# Autodesk Inventor assembly: main climber
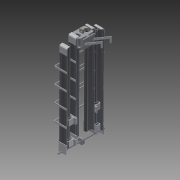
[picture p0: Inventor's stored thumbnail of the model, 180x180]
Saved by Autodesk Inventor 2013 (Build 170138000, 138)
## iProperties
Created: 2013-01-25
Part Number: main climber
Document SubType Name: Assembly
Designer: Arpan
Mass: 3339.77 g
Surface Area: 12818.3 cm^2
Volume: 2944.87 cm^3
Density: 1.1341 g/cm^3
Author: Arpan
## Documents named in this file (16)
- C:\Users\Moses\Documents\GitHub\frc2013CAD\Cimber actual\main climber.iam
- C:\Users\Moses\Documents\GitHub\frc2013CAD\Cimber actual\Shaft 26 inch.ipt
- C:\Users\Moses\Documents\GitHub\frc2013CAD\Cimber actual\Bearing Block long style.iam
- C:\Users\Moses\Documents\GitHub\frc2013CAD\Cimber actual\hook mount plate.ipt
- C:\Users\Moses\Documents\GitHub\frc2013CAD\Cimber actual\tie-together tier 1.ipt
- C:\Users\Moses\Documents\GitHub\frc2013CAD\Cimber actual\endstop.ipt
- C:\Users\Moses\Documents\GitHub\frc2013CAD\Cimber actual\hook faceplate.ipt
- C:\Users\Moses\Documents\GitHub\frc2013CAD\Cimber actual\hook.ipt
- C:\Users\Moses\Documents\GitHub\frc2013CAD\Cimber actual\face mount.ipt
- C:\Users\Moses\Documents\GitHub\frc2013CAD\Cimber actual\bearing block short style.iam
- C:\Users\Moses\Documents\GitHub\frc2013CAD\Cimber actual\upper face mount.ipt
- C:\Users\Moses\Documents\GitHub\frc2013CAD\Cimber actual\tie-together tier 2.ipt
- C:\Users\Moses\Documents\GitHub\frc2013CAD\Cimber actual\arm mout.ipt
- C:\Users\Moses\Documents\GitHub\frc2013CAD\Cimber actual\14 inch shaft.ipt
- C:\Users\Moses\Documents\GitHub\frc2013CAD\Cimber actual\rough pulley.ipt
- C:\Users\Moses\Documents\GitHub\frc2013CAD\Cimber actual\hook mount plate 2.ipt
## Components (34 placed, 15 different names)
1. Shaft 26 inch:1 — Flush:1, Angle:1, Mate:2, Flush:2, Angle:2, Mate:12, Mate:13, Mate:25, Mate:26, Mate:27, Mate:28, Mate:29, Mate:30, Mate:31, Mate:32, Mate:33, Mate:38, Mate:39, Mate:40, Mate:46, Mate:53, Mate:54, Mate:55
2. Shaft 26 inch:2 — Flush:1, Angle:1, Mate:1, Flush:2, Flush:7, Mate:10, Mate:11, Mate:37, Flush:15, Flush:16, Mate:48, Mate:50, Mate:51, Mate:52
3. Bearing Block long style:1 [sub-assembly] — Mate:1, Mate:3, Flush:3
4. Bearing Block long style:2 [sub-assembly] — Mate:2, Mate:3, Angle:2, Flush:3, Mate:98, Flush:25, Flush:26
5. hook mount plate:1 — Mate:98, Mate:99, Flush:25, Flush:26, Flush:27, Mate:100, Flush:28, Mate:101, Flush:29
6. endstop:1 — Mate:12, Mate:13, Mate:46
7. endstop:2 — Flush:7, Mate:10, Mate:11
8. hook faceplate:1 — Mate:20, Mate:21, Mate:22, Flush:13, Flush:14, Mate:23, Mate:99, Mate:101, Flush:29, Mate:102, Flush:30
9. hook:1 — Mate:22, Flush:14, Mate:102
10. hook:2 — Mate:20, Mate:21, Flush:13, Mate:23
11. tie-together tier 1:1 — Mate:25, Mate:26, Mate:27
12. tie-together tier 1:2 — Mate:28, Mate:29, Mate:30
13. tie-together tier 1:3 — Mate:31, Mate:32, Mate:33
14. face mount:1 — Mate:37, Flush:15, Flush:16, Mate:43, Mate:84, Mate:85
15. face mount:2 — Mate:38, Mate:39, Mate:40, Flush:17, Mate:41, Flush:18
16. bearing block short style:1 [sub-assembly] — Flush:17, Mate:41, Flush:18
17. bearing block short style:2 [sub-assembly] — Mate:43, Flush:19, Mate:49, Mate:84, Mate:85, Flush:23
18. bearing block short style:3 [sub-assembly] — Mate:57, Mate:58, Mate:59, Mate:60, Mate:64, Angle:3
19. bearing block short style:4 [sub-assembly] — Mate:48, Flush:19, Mate:49, Mate:65
20. upper face mount:1 — Mate:50, Mate:51, Mate:52
21. upper face mount:2 — Mate:53, Mate:54, Mate:55, Mate:57, Mate:58, Mate:59, Mate:60
22. Shaft 26 inch:3 — Mate:65, Angle:4, Flush:20, Mate:67, Mate:68, Flush:22, Mate:78, Mate:79, Mate:80, Mate:82, Mate:83, Flush:23, Mate:88, Mate:89
23. Shaft 26 inch:4 — Mate:64, Angle:3, Angle:4, Flush:20, Mate:69, Mate:70, Mate:71, Mate:76, Mate:77, Mate:86, Mate:87, Mate:90, Mate:91, Mate:97
24. endstop:3 — Mate:67, Mate:68, Flush:22
25. endstop:4 — Mate:69, Mate:70, Mate:71
26. tie-together tier 2:2 — Mate:76, Mate:77, Mate:78
27. tie-together tier 2:3 — Mate:79, Mate:80
28. tie-together tier 2:4 — Mate:82, Mate:83
29. tie-together tier 2:5 — Mate:86, Mate:87
30. arm mout:1 — Mate:90, Mate:91, Mate:92, Mate:97
31. arm mout:2 — Mate:88, Mate:89, Flush:24, Mate:96
32. 14 inch shaft:1 — Mate:92, Flush:24, Mate:93
33. rough pulley:1 — Mate:93, Mate:96
34. hook mount plate 2:1 — Flush:27, Mate:100, Flush:28, Flush:30
## Relationships (95: Mate 70, Flush 21, Angle 4)
- Flush:1: Shaft 26 inch:1 ↔ Shaft 26 inch:2
- Angle:1 (180 deg): Shaft 26 inch:1 ↔ Shaft 26 inch:2
- Mate:1: Shaft 26 inch:2 ↔ Bearing Block long style:1
- Mate:2: Shaft 26 inch:1 ↔ Bearing Block long style:2
- Mate:3 (12.7 mm): Bearing Block long style:1 ↔ Bearing Block long style:2
- Flush:2: Shaft 26 inch:1 ↔ Shaft 26 inch:2
- Angle:2 (0 deg): Shaft 26 inch:1 ↔ Bearing Block long style:2
- Flush:3: Bearing Block long style:1 ↔ Bearing Block long style:2
- Flush:7: Shaft 26 inch:2 ↔ endstop:2
- Mate:10: Shaft 26 inch:2 ↔ endstop:2
- Mate:11: Shaft 26 inch:2 ↔ endstop:2
- Mate:12: Shaft 26 inch:1 ↔ endstop:1
- Mate:13: Shaft 26 inch:1 ↔ endstop:1
- Mate:20: hook faceplate:1 ↔ hook:2
- Mate:21 (-26.1747 mm): hook faceplate:1 ↔ hook:2
- Mate:22 (26.1874 mm): hook faceplate:1 ↔ hook:1
- Flush:13 (6.35 mm): hook faceplate:1 ↔ hook:2
- Flush:14 (6.35 mm): hook faceplate:1 ↔ hook:1
- Mate:23 (26.1658 mm): hook faceplate:1 ↔ hook:2
- Mate:25: Shaft 26 inch:1 ↔ tie-together tier 1:1
- Mate:26: Shaft 26 inch:1 ↔ tie-together tier 1:1
- Mate:27: Shaft 26 inch:1 ↔ tie-together tier 1:1
- Mate:28: Shaft 26 inch:1 ↔ tie-together tier 1:2
- Mate:29: Shaft 26 inch:1 ↔ tie-together tier 1:2
- Mate:30: Shaft 26 inch:1 ↔ tie-together tier 1:2
- Mate:31: Shaft 26 inch:1 ↔ tie-together tier 1:3
- Mate:32: Shaft 26 inch:1 ↔ tie-together tier 1:3
- Mate:33: Shaft 26 inch:1 ↔ tie-together tier 1:3
- Mate:37: Shaft 26 inch:2 ↔ face mount:1
- Mate:38: Shaft 26 inch:1 ↔ face mount:2
- Flush:15 (-15.24 mm): Shaft 26 inch:2 ↔ face mount:1
- Flush:16 (-12.688 mm): Shaft 26 inch:2 ↔ face mount:1
- Mate:39: Shaft 26 inch:1 ↔ face mount:2
- Mate:40: Shaft 26 inch:1 ↔ face mount:2
- Flush:17 (-12.0142 mm): face mount:2 ↔ bearing block short style:1
- Mate:41: face mount:2 ↔ bearing block short style:1
- Flush:18 (1.1988 mm): face mount:2 ↔ bearing block short style:1
- Mate:43: face mount:1 ↔ bearing block short style:2
- Mate:46: Shaft 26 inch:1 ↔ endstop:1
- Mate:48 (3.175 mm): Shaft 26 inch:2 ↔ bearing block short style:4
- Flush:19: bearing block short style:2 ↔ bearing block short style:4
- Mate:49 (81.698 mm): bearing block short style:2 ↔ bearing block short style:4
- Mate:50: Shaft 26 inch:2 ↔ upper face mount:1
- Mate:51: Shaft 26 inch:2 ↔ upper face mount:1
- Mate:52: Shaft 26 inch:2 ↔ upper face mount:1
- Mate:53: Shaft 26 inch:1 ↔ upper face mount:2
- Mate:54: Shaft 26 inch:1 ↔ upper face mount:2
- Mate:55: Shaft 26 inch:1 ↔ upper face mount:2
- Mate:57: bearing block short style:3 ↔ upper face mount:2
- Mate:58: bearing block short style:3 ↔ upper face mount:2
- Mate:59: bearing block short style:3 ↔ upper face mount:2
- Mate:60: bearing block short style:3 ↔ upper face mount:2
- Mate:64: bearing block short style:3 ↔ Shaft 26 inch:4
- Mate:65: bearing block short style:4 ↔ Shaft 26 inch:3
- Angle:3 (180 deg): bearing block short style:3 ↔ Shaft 26 inch:4
- Angle:4 (180 deg): Shaft 26 inch:3 ↔ Shaft 26 inch:4
- Flush:20: Shaft 26 inch:3 ↔ Shaft 26 inch:4
- Mate:67: Shaft 26 inch:3 ↔ endstop:3
- Mate:68: Shaft 26 inch:3 ↔ endstop:3
- Flush:22: Shaft 26 inch:3 ↔ endstop:3
- Mate:69: Shaft 26 inch:4 ↔ endstop:4
- Mate:70: Shaft 26 inch:4 ↔ endstop:4
- Mate:71: Shaft 26 inch:4 ↔ endstop:4
- Mate:76: Shaft 26 inch:4 ↔ tie-together tier 2:2
- Mate:77: Shaft 26 inch:4 ↔ tie-together tier 2:2
- Mate:78: Shaft 26 inch:3 ↔ tie-together tier 2:2
- Mate:79: Shaft 26 inch:3 ↔ tie-together tier 2:3
- Mate:80: Shaft 26 inch:3 ↔ tie-together tier 2:3
- Mate:82: Shaft 26 inch:3 ↔ tie-together tier 2:4
- Mate:83: Shaft 26 inch:3 ↔ tie-together tier 2:4
- Mate:84: face mount:1 ↔ bearing block short style:2
- Mate:85: face mount:1 ↔ bearing block short style:2
- Flush:23: bearing block short style:2 ↔ Shaft 26 inch:3
- Mate:86: Shaft 26 inch:4 ↔ tie-together tier 2:5
- Mate:87: Shaft 26 inch:4 ↔ tie-together tier 2:5
- Mate:88: Shaft 26 inch:3 ↔ arm mout:2
- Mate:89: Shaft 26 inch:3 ↔ arm mout:2
- Mate:90: Shaft 26 inch:4 ↔ arm mout:1
- Mate:91: Shaft 26 inch:4 ↔ arm mout:1
- Mate:92: arm mout:1 ↔ 14 inch shaft:1
- Flush:24 (-33.1 mm): arm mout:2 ↔ 14 inch shaft:1
- Mate:93: 14 inch shaft:1 ↔ rough pulley:1
- Mate:96 (135.1788 mm): arm mout:2 ↔ rough pulley:1
- Mate:97: Shaft 26 inch:4 ↔ arm mout:1
- Mate:98: Bearing Block long style:2 ↔ hook mount plate:1
- Mate:99: hook mount plate:1 ↔ hook faceplate:1
- Flush:25: Bearing Block long style:2 ↔ hook mount plate:1
- Flush:26 (-12.7 mm): Bearing Block long style:2 ↔ hook mount plate:1
- Flush:27: hook mount plate:1 ↔ hook mount plate 2:1
- Mate:100: hook mount plate:1 ↔ hook mount plate 2:1
- Flush:28: hook mount plate:1 ↔ hook mount plate 2:1
- Mate:101: hook mount plate:1 ↔ hook faceplate:1
- Flush:29: hook mount plate:1 ↔ hook faceplate:1
- Mate:102: hook faceplate:1 ↔ hook:1
- Flush:30 (-38.1 mm): hook faceplate:1 ↔ hook mount plate 2:1
